# Autodesk Inventor assembly: Schachcomputer mit Display
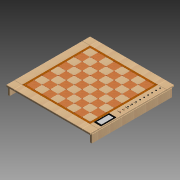
[picture p0: Inventor's stored thumbnail of the model, 180x180]
Saved by Autodesk Inventor 2013 SP1 (Build 170176100, 176)
## iProperties
Created: 2012-12-07
Part Number: Schachcomputer mit Display
Document SubType Name: Assembly
Designer: Sebastian
Author: Sebastian
## Documents named in this file (13)
- E:\Projects\chess\construction\Schachcomputer mit Display.iam
- E:\Projects\chess\construction\Spielfeld.ipt
- E:\Projects\chess\construction\LED.ipt
- E:\Projects\chess\construction\Platine.ipt
- E:\Projects\chess\construction\Rahmen.ipt
- E:\Projects\chess\construction\Wände.ipt
- E:\Projects\chess\construction\Raspberry.ipt
- E:\Projects\chess\construction\Pushbutton.ipt
- E:\Projects\chess\construction\Schalterhalterung.ipt
- E:\Projects\chess\construction\Pin.ipt
- E:\Projects\chess\construction\Hohlstecker.ipt
- E:\Projects\chess\construction\RJ45-Buchse.ipt
- E:\Projects\chess\construction\Display.ipt
## Components (139 placed, 12 different names)
1. Spielfeld:1 — Einfügen:4
2. Platine:1
3. Wände:1
4. Rahmen:1 — Einfügen:1, Einfügen:2, Einfügen:3
5. Raspberry:1
6. LED:82 — Einfügen:2
7. LED:83 — Einfügen:3
8. Schalterhalterung:1
9. Hohlstecker:1
10. RJ45-Buchse:1
11. Display:1
12. LED:1 — Einfügen:4
13. LED:2
14. LED:3
15. LED:4
16. LED:5
17. LED:6
18. LED:7
19. LED:8
20. LED:9
21. LED:10
22. LED:11
23. LED:12
24. LED:13
25. LED:14
26. LED:15
27. LED:16
28. LED:17
29. LED:18
30. LED:19
31. LED:20
32. LED:21
33. LED:22
34. LED:23
35. LED:24
36. LED:25
37. LED:26
38. LED:27
39. LED:28
40. LED:29
41. LED:30
42. LED:31
43. LED:32
44. LED:33
45. LED:34
46. LED:35
47. LED:36
48. LED:37
49. LED:38
50. LED:39
51. LED:40
52. LED:41
53. LED:42
54. LED:43
55. LED:44
56. LED:45
57. LED:46
58. LED:47
59. LED:48
60. LED:49
61. LED:50
62. LED:51
63. LED:52
64. LED:53
65. LED:54
66. LED:55
67. LED:56
68. LED:57
69. LED:58
70. LED:59
71. LED:60
72. LED:61
73. LED:62
74. LED:63
75. LED:64
76. LED:65
77. LED:66
78. LED:67
79. LED:68
80. LED:69
81. LED:70
82. LED:71
83. LED:72
84. LED:73
85. LED:74
86. LED:75
87. LED:76
88. LED:77
89. LED:78
90. LED:79
91. LED:80
92. LED:81
93. Pushbutton:11 — Einfügen:1
94. Pushbutton:12
95. Pushbutton:13
96. Pushbutton:14
97. Pushbutton:15
98. Pushbutton:16
99. Pushbutton:17
100. Pushbutton:18
101. Pushbutton:19
102. Pin:1
103. Pin:2
104. Pin:3
105. Pin:4
106. Pin:5
107. Pin:6
108. Pin:7
109. Pin:8
110. Pin:9
111. Pin:10
112. Pin:11
113. Pin:12
114. Pin:13
115. Pin:14
116. Pin:15
117. Pin:16
118. Pin:17
119. Pin:18
120. Pin:19
121. Pin:20
122. Pin:21
123. Pin:22
124. Pin:23
125. Pin:24
126. Pin:25
127. Pin:26
128. Pin:27
129. Pin:28
130. Pin:29
131. Pin:30
132. Pin:31
133. Pin:32
134. Pin:33
135. Pin:34
136. Pin:35
137. Pin:36
138. Pin:37
139. Pin:38
## Component patterns: Komponentenanordnung LEDs (81 elements), Komponentenanordnung Schalter (9 elements), Komponentenanordnung Stiftleiste oben (13 elements), Komponentenanordnung Stiftleiste rechts (25 elements)
## Relationships (4: Insert 4)
- Einfügen:1 [Insert] (-10 mm): Rahmen:1 ↔ Pushbutton:11
- Einfügen:2 [Insert] (-6.5 mm): Rahmen:1 ↔ LED:82
- Einfügen:3 [Insert] (-6.5 mm): Rahmen:1 ↔ LED:83
- Einfügen:4 [Insert] (0.5 mm): Spielfeld:1 ↔ LED:1
